# Autodesk Inventor assembly: green-house
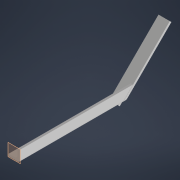
[picture p0: Inventor's stored thumbnail of the model, 180x180]
Saved by Autodesk Inventor 2021 (Build 250183000, 183)
## iProperties
Created: 2020-05-07
Part Number: green-house
Document SubType Name: Assembly
Designer: Jonathan
Author: Jonathan
## Documents named in this file (3)
- C:\Users\Jonathan\green-house\green-house.iam
- C:\Users\Jonathan\Documents\3D_models\Part1.ipt
- C:\Users\Jonathan\Documents\3D_models\Part3.ipt
## Components (2 placed, 2 different names)
1. Frame — Flush:1, Flush:2
2. Part3:1 — Flush:1, Flush:2
## Relationships (2: Flush 2)
- Flush:1: Frame ↔ Part3:1
- Flush:2: Frame ↔ Part3:1
